# Autodesk Inventor assembly: Fan Front
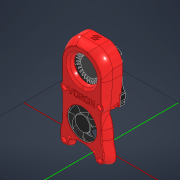
[picture p0: Inventor's stored thumbnail of the model, 180x180]
Saved by Autodesk Inventor 2022.2 (Build 262287010, 287A)
## iProperties
Created: 2022-03-16
Part Number: Fan Front
Document SubType Name: Assembly
Designer: sleib
Author: sleib
## Documents named in this file (7)
- C:\Users\sleib\Projekte\Voron-2\CAD\Inventor\Afterburner\Fan Front.iam
- C:\Users\sleib\Projekte\Voron-2\CAD\Inventor\Afterburner\Fan Front.ipt
- C:\Users\sleib\Projekte\Voron-2\CAD\Inventor\Afterburner\Fan 4040.ipt
- C:\Users\sleib\Projekte\Voron-2\CAD\Inventor\Afterburner\Fan 5015 (stripped).iam
- C:\Users\sleib\Projekte\Voron-2\CAD\Inventor\Afterburner\Fan Spring.ipt
- C:\Users\sleib\Projekte\Voron-2\CAD\Inventor\Afterburner\Fan Back.ipt
- C:\Users\sleib\Projekte\Voron-2\CAD\Inventor\Afterburner\Spacer v1.ipt
## Components (6 placed, 6 different names)
1. Fan Front:1 — Fluchtend:1, Fluchtend:2, Passend:1, Passend:2, Fluchtend:3, Passend:3, Passend:4, Tangential:1, Tangential:2, Passend:5, Tangential:3, Passend:6, Passend:7, Passend:8, Passend:9, Passend:10
2. Fan 4040:1 — Passend:2, Fluchtend:3, Passend:3
3. Fan 5015 (stripped):1 [sub-assembly] — Passend:4, Tangential:1, Tangential:2, Tangential:4
4. Fan Spring:1 — Passend:5, Tangential:3, Tangential:4
5. Fan Back:1 — Passend:6, Passend:7, Passend:8, Passend:11
6. Spacer v1:1 — Passend:9, Passend:10, Passend:11
## Relationships (18: Mate 11, Tangent 4, Flush 3)
- Fluchtend:1 [Flush]: Fan Front:1
- Fluchtend:2 [Flush]: Fan Front:1
- Passend:1 [Mate]: Fan Front:1
- Passend:2 [Mate]: Fan Front:1 ↔ Fan 4040:1
- Fluchtend:3 [Flush]: Fan Front:1 ↔ Fan 4040:1
- Passend:3 [Mate]: Fan Front:1 ↔ Fan 4040:1
- Passend:4 [Mate]: Fan Front:1 ↔ Fan 5015 (stripped):1
- Tangential:1: Fan Front:1 ↔ Fan 5015 (stripped):1
- Tangential:2: Fan Front:1 ↔ Fan 5015 (stripped):1
- Passend:5 [Mate]: Fan Front:1 ↔ Fan Spring:1
- Tangential:3: Fan Front:1 ↔ Fan Spring:1
- Tangential:4: Fan 5015 (stripped):1 ↔ Fan Spring:1
- Passend:6 [Mate]: Fan Front:1 ↔ Fan Back:1
- Passend:7 [Mate]: Fan Front:1 ↔ Fan Back:1
- Passend:8 [Mate]: Fan Front:1 ↔ Fan Back:1
- Passend:9 [Mate]: Fan Front:1 ↔ Spacer v1:1
- Passend:10 [Mate]: Fan Front:1 ↔ Spacer v1:1
- Passend:11 [Mate]: Fan Back:1 ↔ Spacer v1:1
